# Autodesk Inventor assembly: Ensamble Dispensador V2
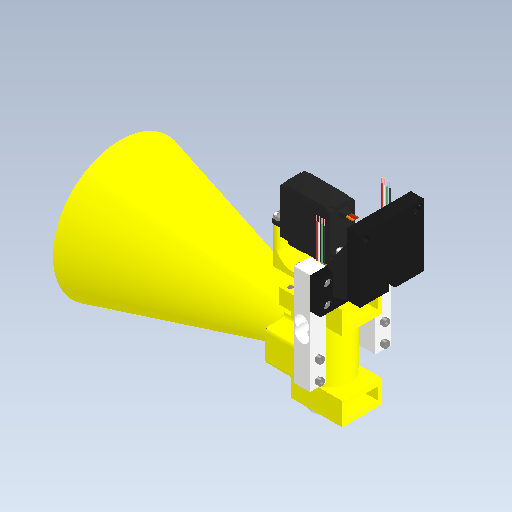
[picture p0: Inventor's stored thumbnail of the model, 512x512]
Saved by Autodesk Inventor 2020.3 (Build 243373000, 373)
## iProperties
Created: 2020-08-17
Part Number: Ensamble Dispensador V2
Document SubType Name: Assembly
Designer: juanp
Mass: 289.664 g
Surface Area: 1896.22 cm^2
Volume: 247.739 cm^3
Density: 1.16923 g/cm^3
Author: juanp
## Documents named in this file (15)
- C:\Users\juanp\Desktop\Robocol\Diseño EVA\Dispensador\Ensamble Dispensador V2.iam
- C:\Users\juanp\Desktop\Robocol\Diseño EVA\Dispensador\Tornillo.ipt
- C:\Users\juanp\Desktop\Robocol\Diseño EVA\Dispensador\Tubo.ipt
- C:\Users\juanp\Desktop\Robocol\Diseño EVA\Dispensador\Dud rodamiento.ipt
- C:\Users\juanp\Desktop\Robocol\Diseño EVA\Dispensador\Acoplador Eje.ipt
- C:\Users\juanp\Desktop\Robocol\Diseño EVA\Dispensador\CELDA DE PRESION ARDUINO.ipt
- C:\Users\juanp\Desktop\Robocol\Diseño EVA\Dispensador\Servo MG996R\Servo Motor MG996R.iam
- C:\Users\juanp\Documents\Inventor\Content Center Files\R2020\en-US\ANSI B 18.2.4.1 M(1)\ANSI B 18.2.4.1 M - M3 x 0.5Style 1.ipt
- C:\Users\juanp\Documents\Inventor\Content Center Files\R2020\en-US\ANSI B 18.2.4.1 M(1)\ANSI B 18.2.4.1 M - M2 x 0.4Style 1.ipt
- C:\Users\juanp\Desktop\Robocol\Diseño EVA\Dispensador\Soporte.ipt
- C:\Users\juanp\Documents\Inventor\Content Center Files\R2020\en-US\ANSI B18.3.1M(6)\ANSI B18.3.1M - M2x0.4 x 12(1).ipt
- C:\Users\juanp\Desktop\Robocol\Diseño EVA\Dispensador\Adaptador Acoplador.ipt
- C:\Users\juanp\Documents\Inventor\Content Center Files\R2020\en-US\ANSI B18.3.1M(1)\ANSI B18.3.1M - M3x0.5 x 40(2).ipt
- C:\Users\juanp\Documents\Inventor\Content Center Files\R2020\en-US\ANSI B18.3.1M(1)\ANSI B18.3.1M - M3x0.5 x 20(2).ipt
- C:\Users\juanp\Documents\Inventor\Content Center Files\R2020\en-US\ANSI B18.6.7M(00)\ANSI B18.6.7M - M4x0.7 x 5(4).ipt
## Components (38 placed, 14 different names)
1. Tornillo:1 — Mate:1, Mate:2, Mate:13, Angle:11, Mate:81, Mate:83
2. Tubo:1 — Mate:1, Mate:2, Flush:1, Mate:6, Flush:2, Mate:10, Mate:11, Mate:12, Mate:14, Mate:15, Mate:16, Angle:1, Mate:24, Mate:25, Mate:26, Mate:27, Angle:5, Mate:33, Mate:70, Mate:71, Mate:72, Mate:73, Mate:74, Mate:75, Mate:82
3. Dud rodamiento:1 — Flush:1, Mate:83
4. Dud rodamiento:2 — Mate:6, Flush:2
5. CELDA DE PRESION ARDUINO:1 — Mate:10, Mate:11, Mate:12, Mate:53, Mate:62, Mate:63
6. CELDA DE PRESION ARDUINO:2 — Mate:14, Mate:15, Mate:16, Mate:28, Mate:54, Mate:55, Mate:60, Mate:61, Mate:64
7. Servo Motor MG996R:1 [sub-assembly] — Mate:13, Angle:1, Mate:47, Mate:50, Mate:76, Mate:77, Mate:78, Mate:79, Mate:80, Mate:82
8. Broached Socket Head Cap Screw - Metric M3x0.5 x 40:3 — Mate:24, Flush:3, Mate:29
9. Hex Nut Metric M3 x 0.5:1 — Mate:29, Flush:8, Angle:4
10. Broached Socket Head Cap Screw - Metric M3x0.5 x 40:1 — Mate:27, Flush:5, Mate:32
11. Broached Socket Head Cap Screw - Metric M3x0.5 x 40:2 — Mate:26, Flush:4, Flush:5, Mate:28, Mate:31
12. Broached Socket Head Cap Screw - Metric M3x0.5 x 40:4 — Mate:25, Flush:3, Flush:4, Mate:30
13. Hex Nut Metric M3 x 0.5:2 — Mate:31, Flush:6, Angle:2, Angle:3
14. Hex Nut Metric M3 x 0.5:3 — Mate:32, Flush:6, Flush:7, Angle:2, Mate:33
15. Hex Nut Metric M3 x 0.5:4 — Mate:30, Flush:7, Flush:8, Angle:3, Angle:4, Angle:5
16. Forged Socket Head Cap Screw - Metric M2x0.4 x 12:4 — Flush:23, Mate:66, Mate:70
17. Hex Nut Metric M2 x 0.4:3 — Flush:28, Mate:66, Angle:16, Angle:17, Mate:74
18. Soporte:1 — Mate:53, Mate:54, Mate:55, Mate:65, Angle:15
19. Acoplador Eje:1 — Mate:47, Mate:50, Mate:51, Angle:10
20. Adaptador Acoplador:1 — Mate:51, Angle:10, Angle:11, Mate:81
21. Hex Nut Metric M3 x 0.5:5 — Flush:21, Mate:57, Angle:14
22. Hex Nut Metric M3 x 0.5:6 — Flush:20, Flush:21, Mate:58, Angle:12, Angle:13, Mate:65, Angle:15
23. Hex Nut Metric M3 x 0.5:7 — Flush:19, Mate:56, Angle:13, Angle:14
24. Hex Nut Metric M3 x 0.5:8 — Flush:19, Flush:20, Mate:59, Angle:12
25. Broached Socket Head Cap Screw - Metric M3x0.5 x 20:2 — Flush:16, Flush:17, Flush:18, Mate:59, Mate:61
26. Broached Socket Head Cap Screw - Metric M3x0.5 x 20:4 — Flush:16, Flush:17, Mate:57, Mate:63, Flush:22
27. Broached Socket Head Cap Screw - Metric M3x0.5 x 20:3 — Mate:56, Mate:62, Flush:22
28. Broached Socket Head Cap Screw - Metric M3x0.5 x 20:1 — Flush:18, Mate:58, Mate:60, Mate:64
29. Forged Socket Head Cap Screw - Metric M2x0.4 x 12:5 — Flush:23, Flush:24, Mate:67, Mate:71, Mate:75
30. Forged Socket Head Cap Screw - Metric M2x0.4 x 12:6 — Flush:24, Flush:25, Mate:69, Mate:72
31. Forged Socket Head Cap Screw - Metric M2x0.4 x 12:7 — Flush:25, Mate:68, Mate:73
32. Hex Nut Metric M2 x 0.4:4 — Flush:27, Flush:28, Mate:67, Angle:16
33. Hex Nut Metric M2 x 0.4:5 — Flush:26, Flush:27, Mate:68, Angle:18
34. Hex Nut Metric M2 x 0.4:6 — Flush:26, Mate:69, Angle:17, Angle:18
35. Cross Recessed Pan Head Machine Screw - Type I - Metric M4x0.7 x 5:2 — Mate:76, Flush:29
36. Cross Recessed Pan Head Machine Screw - Type I - Metric M4x0.7 x 5:3 — Flush:29, Flush:30, Mate:79
37. Cross Recessed Pan Head Machine Screw - Type I - Metric M4x0.7 x 5:4 — Flush:30, Flush:31, Mate:78
38. Cross Recessed Pan Head Machine Screw - Type I - Metric M4x0.7 x 5:1 — Flush:31, Mate:77, Mate:80
## Relationships (92: Mate 54, Flush 24, Angle 14)
- Mate:1: Tornillo:1 ↔ Tubo:1
- Mate:2: Tornillo:1 ↔ Tubo:1
- Flush:1: Tubo:1 ↔ Dud rodamiento:1
- Mate:6: Tubo:1 ↔ Dud rodamiento:2
- Flush:2: Tubo:1 ↔ Dud rodamiento:2
- Mate:10: Tubo:1 ↔ CELDA DE PRESION ARDUINO:1
- Mate:11: Tubo:1 ↔ CELDA DE PRESION ARDUINO:1
- Mate:12: Tubo:1 ↔ CELDA DE PRESION ARDUINO:1
- Mate:13: Tornillo:1 ↔ Servo Motor MG996R:1
- Mate:14: Tubo:1 ↔ CELDA DE PRESION ARDUINO:2
- Mate:15: Tubo:1 ↔ CELDA DE PRESION ARDUINO:2
- Mate:16: Tubo:1 ↔ CELDA DE PRESION ARDUINO:2
- Angle:1 (0 deg): Tubo:1 ↔ Servo Motor MG996R:1
- Mate:24: Tubo:1 ↔ Broached Socket Head Cap Screw - Metric M3x0.5 x 40:3
- Mate:25: Tubo:1 ↔ Broached Socket Head Cap Screw - Metric M3x0.5 x 40:4
- Mate:26: Tubo:1 ↔ Broached Socket Head Cap Screw - Metric M3x0.5 x 40:2
- Mate:27: Tubo:1 ↔ Broached Socket Head Cap Screw - Metric M3x0.5 x 40:1
- Flush:3: Broached Socket Head Cap Screw - Metric M3x0.5 x 40:3 ↔ Broached Socket Head Cap Screw - Metric M3x0.5 x 40:4
- Flush:4: Broached Socket Head Cap Screw - Metric M3x0.5 x 40:2 ↔ Broached Socket Head Cap Screw - Metric M3x0.5 x 40:4
- Flush:5: Broached Socket Head Cap Screw - Metric M3x0.5 x 40:1 ↔ Broached Socket Head Cap Screw - Metric M3x0.5 x 40:2
- Mate:28: CELDA DE PRESION ARDUINO:2 ↔ Broached Socket Head Cap Screw - Metric M3x0.5 x 40:2
- Mate:29: Broached Socket Head Cap Screw - Metric M3x0.5 x 40:3 ↔ Hex Nut Metric M3 x 0.5:1
- Mate:30: Broached Socket Head Cap Screw - Metric M3x0.5 x 40:4 ↔ Hex Nut Metric M3 x 0.5:4
- Mate:31: Broached Socket Head Cap Screw - Metric M3x0.5 x 40:2 ↔ Hex Nut Metric M3 x 0.5:2
- Mate:32: Broached Socket Head Cap Screw - Metric M3x0.5 x 40:1 ↔ Hex Nut Metric M3 x 0.5:3
- Flush:6: Hex Nut Metric M3 x 0.5:2 ↔ Hex Nut Metric M3 x 0.5:3
- Flush:7: Hex Nut Metric M3 x 0.5:3 ↔ Hex Nut Metric M3 x 0.5:4
- Flush:8: Hex Nut Metric M3 x 0.5:1 ↔ Hex Nut Metric M3 x 0.5:4
- Angle:2 (0 deg): Hex Nut Metric M3 x 0.5:2 ↔ Hex Nut Metric M3 x 0.5:3
- Angle:3 (0 deg): Hex Nut Metric M3 x 0.5:2 ↔ Hex Nut Metric M3 x 0.5:4
- Angle:4 (0 deg): Hex Nut Metric M3 x 0.5:1 ↔ Hex Nut Metric M3 x 0.5:4
- Angle:5 (0 deg): Tubo:1 ↔ Hex Nut Metric M3 x 0.5:4
- Mate:33: Tubo:1 ↔ Hex Nut Metric M3 x 0.5:3
- Mate:47: Servo Motor MG996R:1 ↔ Acoplador Eje:1
- Mate:50: Servo Motor MG996R:1 ↔ Acoplador Eje:1
- Mate:51: Acoplador Eje:1 ↔ Adaptador Acoplador:1
- Angle:10 (0 deg): Acoplador Eje:1 ↔ Adaptador Acoplador:1
- Angle:11 (0 deg): Tornillo:1 ↔ Adaptador Acoplador:1
- Mate:53: CELDA DE PRESION ARDUINO:1 ↔ Soporte:1
- Mate:54: CELDA DE PRESION ARDUINO:2 ↔ Soporte:1
- Mate:55: CELDA DE PRESION ARDUINO:2 ↔ Soporte:1
- Flush:16: Broached Socket Head Cap Screw - Metric M3x0.5 x 20:2 ↔ Broached Socket Head Cap Screw - Metric M3x0.5 x 20:4
- Flush:17: Broached Socket Head Cap Screw - Metric M3x0.5 x 20:2 ↔ Broached Socket Head Cap Screw - Metric M3x0.5 x 20:4
- Flush:18: Broached Socket Head Cap Screw - Metric M3x0.5 x 20:2 ↔ Broached Socket Head Cap Screw - Metric M3x0.5 x 20:1
- Flush:19: Hex Nut Metric M3 x 0.5:7 ↔ Hex Nut Metric M3 x 0.5:8
- Flush:20: Hex Nut Metric M3 x 0.5:6 ↔ Hex Nut Metric M3 x 0.5:8
- Flush:21: Hex Nut Metric M3 x 0.5:5 ↔ Hex Nut Metric M3 x 0.5:6
- Mate:56: Hex Nut Metric M3 x 0.5:7 ↔ Broached Socket Head Cap Screw - Metric M3x0.5 x 20:3
- Mate:57: Hex Nut Metric M3 x 0.5:5 ↔ Broached Socket Head Cap Screw - Metric M3x0.5 x 20:4
- Mate:58: Hex Nut Metric M3 x 0.5:6 ↔ Broached Socket Head Cap Screw - Metric M3x0.5 x 20:1
- Mate:59: Hex Nut Metric M3 x 0.5:8 ↔ Broached Socket Head Cap Screw - Metric M3x0.5 x 20:2
- Angle:12 (0 deg): Hex Nut Metric M3 x 0.5:6 ↔ Hex Nut Metric M3 x 0.5:8
- Angle:13 (0 deg): Hex Nut Metric M3 x 0.5:6 ↔ Hex Nut Metric M3 x 0.5:7
- Angle:14 (0 deg): Hex Nut Metric M3 x 0.5:5 ↔ Hex Nut Metric M3 x 0.5:7
- Mate:60: CELDA DE PRESION ARDUINO:2 ↔ Broached Socket Head Cap Screw - Metric M3x0.5 x 20:1
- Mate:61: CELDA DE PRESION ARDUINO:2 ↔ Broached Socket Head Cap Screw - Metric M3x0.5 x 20:2
- Mate:62: CELDA DE PRESION ARDUINO:1 ↔ Broached Socket Head Cap Screw - Metric M3x0.5 x 20:3
- Mate:63: CELDA DE PRESION ARDUINO:1 ↔ Broached Socket Head Cap Screw - Metric M3x0.5 x 20:4
- Mate:64: CELDA DE PRESION ARDUINO:2 ↔ Broached Socket Head Cap Screw - Metric M3x0.5 x 20:1
- Mate:65: Soporte:1 ↔ Hex Nut Metric M3 x 0.5:6
- Angle:15 (0 deg): Soporte:1 ↔ Hex Nut Metric M3 x 0.5:6
- Flush:22: Broached Socket Head Cap Screw - Metric M3x0.5 x 20:4 ↔ Broached Socket Head Cap Screw - Metric M3x0.5 x 20:3
- Flush:23: Forged Socket Head Cap Screw - Metric M2x0.4 x 12:4 ↔ Forged Socket Head Cap Screw - Metric M2x0.4 x 12:5
- Flush:24: Forged Socket Head Cap Screw - Metric M2x0.4 x 12:5 ↔ Forged Socket Head Cap Screw - Metric M2x0.4 x 12:6
- Flush:25: Forged Socket Head Cap Screw - Metric M2x0.4 x 12:6 ↔ Forged Socket Head Cap Screw - Metric M2x0.4 x 12:7
- Flush:26: Hex Nut Metric M2 x 0.4:5 ↔ Hex Nut Metric M2 x 0.4:6
- Flush:27: Hex Nut Metric M2 x 0.4:4 ↔ Hex Nut Metric M2 x 0.4:5
- Flush:28: Hex Nut Metric M2 x 0.4:3 ↔ Hex Nut Metric M2 x 0.4:4
- Mate:66: Forged Socket Head Cap Screw - Metric M2x0.4 x 12:4 ↔ Hex Nut Metric M2 x 0.4:3
- Mate:67: Forged Socket Head Cap Screw - Metric M2x0.4 x 12:5 ↔ Hex Nut Metric M2 x 0.4:4
- Mate:68: Forged Socket Head Cap Screw - Metric M2x0.4 x 12:7 ↔ Hex Nut Metric M2 x 0.4:5
- Mate:69: Forged Socket Head Cap Screw - Metric M2x0.4 x 12:6 ↔ Hex Nut Metric M2 x 0.4:6
- Mate:70: Tubo:1 ↔ Forged Socket Head Cap Screw - Metric M2x0.4 x 12:4
- Mate:71: Tubo:1 ↔ Forged Socket Head Cap Screw - Metric M2x0.4 x 12:5
- Mate:72: Tubo:1 ↔ Forged Socket Head Cap Screw - Metric M2x0.4 x 12:6
- Mate:73: Tubo:1 ↔ Forged Socket Head Cap Screw - Metric M2x0.4 x 12:7
- Angle:16 (0 deg): Hex Nut Metric M2 x 0.4:3 ↔ Hex Nut Metric M2 x 0.4:4
- Angle:17 (0 deg): Hex Nut Metric M2 x 0.4:3 ↔ Hex Nut Metric M2 x 0.4:6
- Angle:18 (0 deg): Hex Nut Metric M2 x 0.4:5 ↔ Hex Nut Metric M2 x 0.4:6
- Mate:74: Tubo:1 ↔ Hex Nut Metric M2 x 0.4:3
- Mate:75: Tubo:1 ↔ Forged Socket Head Cap Screw - Metric M2x0.4 x 12:5
- Mate:76: Servo Motor MG996R:1 ↔ Cross Recessed Pan Head Machine Screw - Type I - Metric M4x0.7 x 5:2
- Flush:29: Cross Recessed Pan Head Machine Screw - Type I - Metric M4x0.7 x 5:2 ↔ Cross Recessed Pan Head Machine Screw - Type I - Metric M4x0.7 x 5:3
- Flush:30: Cross Recessed Pan Head Machine Screw - Type I - Metric M4x0.7 x 5:3 ↔ Cross Recessed Pan Head Machine Screw - Type I - Metric M4x0.7 x 5:4
- Flush:31: Cross Recessed Pan Head Machine Screw - Type I - Metric M4x0.7 x 5:4 ↔ Cross Recessed Pan Head Machine Screw - Type I - Metric M4x0.7 x 5:1
- Mate:77: Servo Motor MG996R:1 ↔ Cross Recessed Pan Head Machine Screw - Type I - Metric M4x0.7 x 5:1
- Mate:78: Servo Motor MG996R:1 ↔ Cross Recessed Pan Head Machine Screw - Type I - Metric M4x0.7 x 5:4
- Mate:79: Servo Motor MG996R:1 ↔ Cross Recessed Pan Head Machine Screw - Type I - Metric M4x0.7 x 5:3
- Mate:80: Servo Motor MG996R:1 ↔ Cross Recessed Pan Head Machine Screw - Type I - Metric M4x0.7 x 5:1
- Mate:81: Tornillo:1 ↔ Adaptador Acoplador:1
- Mate:82: Tubo:1 ↔ Servo Motor MG996R:1
- Mate:83: Tornillo:1 ↔ Dud rodamiento:1
